# Autodesk Inventor assembly: WheelAssembly_v9
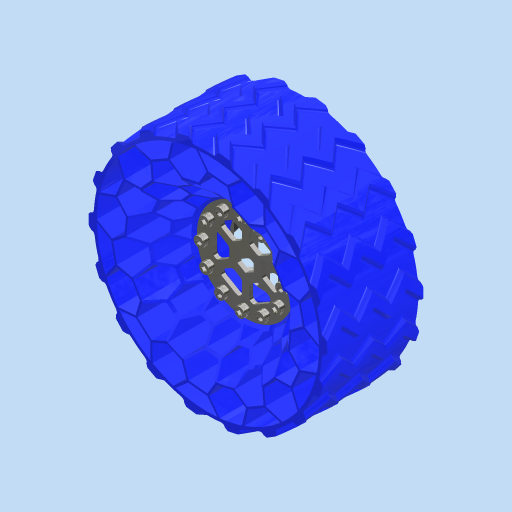
[picture p0: Inventor's stored thumbnail of the model, 512x512]
Saved by Autodesk Inventor 2023 (Build 270158000, 158)
## iProperties
Created: 2023-04-22
Part Number: WheelAssembly_v9
Document SubType Name: Assembly
Designer: asach
Author: asach
## Documents named in this file (5)
- C:\Github\BehrendURC\CAD\Chassis V3\Wheel\WheelAssembly_v9.iam
- C:\Github\BehrendURC\CAD\Chassis V3\Wheel\Tire_v9.ipt
- C:\Github\BehrendURC\CAD\Chassis V3\Wheel\ThickWheelPlate_v8.ipt
- C:\Github\BehrendURC\CAD\Chassis V3\Wheel\WheelPlateBolt_1inch.ipt
- C:\Github\BehrendURC\CAD\Chassis V3\Wheel\WheelPlateNut.ipt
## Components (27 placed, 4 different names)
1. Tire_v9:1 — Mate:1, Mate:2, Mate:3, Mate:4, Mate:5, Mate:6
2. ThickWheelPlate_v8:1 — Mate:1, Mate:2, Mate:3, Mate:7, Mate:8
3. ThickWheelPlate_v8:2 — Mate:4, Mate:5, Mate:6, Mate:9
4. WheelPlateBolt_1inch:1 — Mate:7, Mate:8, Mate:10
5. WheelPlateNut:1 — Mate:9, Mate:10
6. WheelPlateBolt_1inch:2
7. WheelPlateNut:2
8. WheelPlateBolt_1inch:3
9. WheelPlateNut:3
10. WheelPlateBolt_1inch:4
11. WheelPlateNut:4
12. WheelPlateBolt_1inch:5
13. WheelPlateNut:5
14. WheelPlateBolt_1inch:6
15. WheelPlateNut:6
16. WheelPlateBolt_1inch:7
17. WheelPlateNut:7
18. WheelPlateBolt_1inch:8
19. WheelPlateNut:8
20. WheelPlateBolt_1inch:9
21. WheelPlateNut:9
22. WheelPlateBolt_1inch:10
23. WheelPlateNut:10
24. WheelPlateBolt_1inch:11
25. WheelPlateNut:11
26. WheelPlateBolt_1inch:12
27. WheelPlateNut:12
## Component patterns: (12 elements, first: WheelPlateBolt_1inch:1 + WheelPlateNut:1)
## Relationships (10: Mate 10)
- Mate:1: Tire_v9:1 ↔ ThickWheelPlate_v8:1
- Mate:2: Tire_v9:1 ↔ ThickWheelPlate_v8:1
- Mate:3: Tire_v9:1 ↔ ThickWheelPlate_v8:1
- Mate:4: Tire_v9:1 ↔ ThickWheelPlate_v8:2
- Mate:5: Tire_v9:1 ↔ ThickWheelPlate_v8:2
- Mate:6: Tire_v9:1 ↔ ThickWheelPlate_v8:2
- Mate:7: ThickWheelPlate_v8:1 ↔ WheelPlateBolt_1inch:1
- Mate:8: ThickWheelPlate_v8:1 ↔ WheelPlateBolt_1inch:1
- Mate:9: ThickWheelPlate_v8:2 ↔ WheelPlateNut:1
- Mate:10: WheelPlateBolt_1inch:1 ↔ WheelPlateNut:1
